# Autodesk Inventor assembly: working
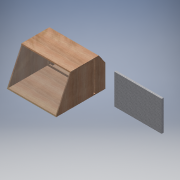
[picture p0: Inventor's stored thumbnail of the model, 180x180]
Saved by Autodesk Inventor 2017 (Build 210142000, 142)
## iProperties
Created: 2019-04-07
Part Number: working
Document SubType Name: Assembly
Designer: Brian
Author: Brian
## Documents named in this file (18)
- B:\Miniatures\spray booth\OldVersions\working.iam
- B:\Miniatures\spray booth\Acrylic Cover.ipt
- B:\Miniatures\spray booth\Filter Frame - Top.ipt
- B:\Miniatures\spray booth\Filter Frame - Bottom.ipt
- B:\Miniatures\spray booth\2x4 - Top Left.ipt
- B:\Miniatures\spray booth\2x4 - Bottom Left.ipt
- B:\Miniatures\spray booth\Filter Frame - Left.ipt
- B:\Miniatures\spray booth\Top Side.ipt
- B:\Miniatures\spray booth\Filter Frame - Right.ipt
- B:\Miniatures\spray booth\Filter.ipt
- B:\Miniatures\spray booth\Back Side.ipt
- B:\Miniatures\spray booth\Right Side - Forward.ipt
- B:\Miniatures\spray booth\Bottom Side.ipt
- B:\Miniatures\spray booth\2x4 - Bottom Right.ipt
- B:\Miniatures\spray booth\2x4 - Top Right.ipt
- B:\Miniatures\spray booth\Right Side - Rear.ipt
- B:\Miniatures\spray booth\Cap Side.ipt
- B:\Miniatures\spray booth\Left Side.ipt
## Components (17 placed, 17 different names)
1. Acrylic Cover:1 — Rotational:1
2. Filter Frame - Top:1
3. Filter Frame - Bottom:1
4. 2x4 - Top Left:1
5. 2x4 - Bottom Left:1
6. Filter Frame - Left:1
7. Top Side:1 — Rotational:1
8. Filter Frame - Right:1
9. Filter:1 — Slider:1
10. Back Side:1
11. Right Side - Forward:1 — Slider:1
12. Bottom Side:1
13. 2x4 - Bottom Right:1
14. 2x4 - Top Right:1
15. Right Side - Rear:1
16. Cap Side:1
17. Left Side:1
## Relationships (2: RevoluteJoint 1, TranslationJoint 1)
- Rotational:1 [RevoluteJoint]: Acrylic Cover:1 ↔ Top Side:1
- Slider:1 [TranslationJoint]: Filter:1 ↔ Right Side - Forward:1
